# Autodesk Inventor assembly: 046-DXP(F,D-166-3)
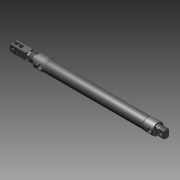
[picture p0: Inventor's stored thumbnail of the model, 180x180]
Saved by Autodesk Inventor 2015 (Build 190159000, 159)
## iProperties
Category: PARTsolutions
Company: BIMBA
Created: 2015-01-31
Part Number: 046-DXP(F,D-166-3)
Catalog Web Link: www.cadenas.de
Description: Original Line Standard Air Cylinders-
Vendor: BIMBA
Document SubType Name: Assembly
Designer: PARTuser1
Manufacturer: BIMBA
PSOL_IDENT_0: {$CADENAS_DATA\23d-libs\bimba\bimba\bimba_imperial\bimba_full_line\original_line_cylinders\standard_
PSOL_IDENT_1: air_cylinders\standard_air_cylinder_asmtab.prj},325 {VTYP=3D},{STYP=ASSTAB},{NB=046-DXP(F,D-166-3)},
PSOL_IDENT_2: {LINA=046-DXP},{NN=Original Line Standard Air Cylinders},{DATE=08.09.2014 04:47:41},{GEOMDATE=08.09.
PSOL_IDENT_3: 2014 04:47:39},{VERSION=},{LINEID=50},{LINESUBID=-1},{WBVAR=STROKE,ACTING,MNT,DER,NR,BM,CO,OO,VO,M,E
PSOL_IDENT_4: E,EEL,K,Q,Y,G,T,B,H,SER,SR,NT,W,HL,STPT1,STPT2,STPT3,STPT4,MB,PB,PRC,TB,MN}  {NB=046-DXP(F,D-166-3)}
PSOL_IDENT_5: ,{LINA=046-DXP},{KT=DUMMY},{PN=046-DXP},{PNC=046-DXP(F,D-166-3)},{PNA=(D-166-3)},{DASH=-},{BORE1=0.7
PSOL_IDENT_6: 5000000},{BORE=3/4\" (04)},{BOREPN=04},{STROKE=6.000},{STROKEALG=[0.011:50/0.001]},{STROKE1=6.000},{
PSOL_IDENT_7: ACTING=D},{ACTINGALG= '' , 'Single Acting (SA)' , 'R' , 'Reverse Single Acting (SA)' , 'D' , 'Double
PSOL_IDENT_8: Acting (SA)' },{ACTINGPN=D},{MNT=XP},{MNTALG= '' , 'Front Nose Mounting (SA)' , 'P' , 'Rear Pivot M
PSOL_IDENT_9: ounting (SA)' , 'XP' , 'Double End or Pivot Mounting (SA)' , 'X' , 'Double End Mounting (SA)' , 'BF'
PSOL_IDENT_10: , 'Front Block Mounting (SA)' , 'BR' , 'Rear Block Mounting for Vertical Positioning (SA)' , 'BFT'
PSOL_IDENT_11: , 'Front Block Trunnion Mounting (SA)' , 'BRT' , 'Rear Block Trunnion Mounting (SA)' },{TYPE=},{MNTP
PSOL_IDENT_12: N=XP},{DER=},{DERALG= '' , 'N/A' },{NR=},{NRALG= '' , 'N/A' },{NRPN=},{BM=},{BMALG= '' , 'N/A' },{BM
PSOL_IDENT_13: PN=},{CO=},{COALG= '' , 'N/A' },{OO=},{OOALG= '', 'N/A' },{OOPN=},{VO=Z},{VOALG= 'Z' , 'N/A' },{VOPN=
PSOL_IDENT_14: },{OOVOPN=},{M=},{MALG= '', 'Without Magnet', 'M', 'With Magnet' },{EE=},{EEL=0.000},{EEMAX=44.0000}
PSOL_IDENT_15: ,{EEALG= '', 'Without Extra Extension', 'EE', 'With Extra Extension' },{EELALG=0},{EEPN=},{EEPN1=0.0
PSOL_IDENT_16: 00},{K=},{KALG= '', 'Standard' , 'K' , 'Ports Rotated 90deg K' },{KPN=},{Q=},{QALG= '' , 'N/A' },{QP
PSOL_IDENT_17: N=},{Y=},{YALG= '' , 'Without Pivot Bushing' , 'Y' , 'With Pivot Bushing' },{YPN=},{YCON=},{F=},{FAL
PSOL_IDENT_18: G= '', 'Non-Coated (Standard)', 'F', 'Molycoated' },{FPN=},{G=},{GPN=},{GPN99=},{T=},{TALG= '' , 'St
PSOL_IDENT_19: andard -20° to 200°F (-29° to 95°C)' , 'N' , 'Low Temperature' , 'V' , 'High Temperature' },{NPN=},{
PSOL_IDENT_20: VPN=},{B=},{BALG= '', 'W/out Bumpers' , 'B' , 'W/ Bumpers' },{BPN=},{H=},{HALG= '', 'N/A' },{HPN=},{
PSOL_IDENT_21: SER=},{SERALG= '' , 'Without Spring Extend/Return' , 'JS' , 'With Spring Return' , 'JR' , 'With Spri
PSOL_IDENT_22: ng Extend' },{SR=},{SRALG= '' , 'Standard Stainless Steel' },{SRPN=},{SRCON=0},{NT=},{NTPN=},{W=},{W
PSOL_IDENT_23: ALG= '' , 'Without Wiper' , 'W' , 'With Wiper' },{WPN=},{E=},{EALG= '' , 'Standard Seals/Lube' , 'E'
PSOL_IDENT_24: , 'Non-Lube Seals/Lube' },{EPN=},{HL=},{HLALG= '' , 'Without Low Pressure Hydraulic' , 'HL' , 'With
PSOL_IDENT_25: Low Pressure Hydraulic' },{ST=},{STALG= '' , 'N/A' },{STPT1=},{STPT1ALG= '' , 'N/A' },{STPT2=},{STP
PSOL_IDENT_26: T2ALG= '' , 'N/A' },{STPT3=},{STPT3ALG= '' , 'N/A' },{STPT4=},{STPT4ALG= '' , 'N/A' },{STPN=},{MB=},
PSOL_IDENT_27: {MBALG= '' , 'Without Mounting Bracket' , 'F,D-129' , 'D-129 (front)'  , 'R,D-129' , 'D-129 (rear)'
PSOL_IDENT_28: , '2x,D-129' , 'D-129 (front & rear)'},{MBPN=},{MBPNALL=D-129},{MBPNALLREAR=D-129},{PB=},{PBALG= ''
PSOL_IDENT_29: , 'Without Pivot Bracket' , 'D-13498-A' , 'D-13498-A' },{PBPN=},{PBPNALL=D-13498-A},{PRC=F,D-166-3},
PSOL_IDENT_30: {PRCALG= '' , 'W/out Pivot Rod Clevis' , 'F,D-166-3' , 'D-166-3 (front)' },{PRCPN=(F,D-166-3)},{PRCP
PSOL_IDENT_31: NALL=D-166-3},{TB=},{TBALG= '' , 'N/A' },{TBPN=},{TBPNALL=},{MN=},{MNALG= '' , 'N/A' },{MNPN=},{MNCO
PSOL_IDENT_32: NF=},{MNCONR=},{TLEN=7.2555},{FRAC=44.7500},{RGCON=},{RGDACCON=R},{RHCON=P},{RHCON1=P},{RHCONON=1},{
PSOL_IDENT_33: RHACCON=},{FNUTCON=1},{RNUTCON=1},{FNUTPN=D-9},{RNUTPN=D-9},{FNUTTRANS=0.0000},{RNUTTRANS=0.0000},{V
PSOL_IDENT_34: HOLECON=0},{A1=1.5940},{A1N=0.8750},{A1P=1.5940},{A1B=1.5940},{A4=0.2525},{A4N=0.3130},{A4P=0.2525},
PSOL_IDENT_35: {A5=0.0300},{A1H=1.594},{A1NH=0.5310},{A1PH=1.5940},{A1BH=1.0940},{A1SH=1.2190},{A2H=0.2190},{A2NH=0
PSOL_IDENT_36: .2190},{LENGTH=3.7500},{LENGTH1=3.7500},{LENGTH2=3.8100},{MUL=6.0000},{MUL11=6.0000},{MUL22=16.14},{
PSOL_IDENT_37: MUL33=10.1400},{MUL2=6.0000},{MUL211=6.0000},{MUL222=2.6900},{MUL233=1.6900},{SSS=12.0000},{RGLEN=1.
PSOL_IDENT_38: 3715},{RHLEN=1.1230},{SSS1=7.0000},{A13=1.3120},{DIF=0.0000},{G5=0.6250},{ON=0},{SSADD=0.0000},{BADD=
PSOL_IDENT_39: 0.0000},{MADD=0.0000},{NVADD=0.0000},{TRACKL=6.9655},{TRACKCON=D-74168},{TRIMCON=0},{TRIMCON1=0},{PI
PSOL_IDENT_40: NCON=D-51},{FSPACE=0.7783},{SPACE=0.1071},{TEXT=0.1875},{S1=1.0000},{D1=0.8325},{D1N=0.8050},{D1B=0.
PSOL_IDENT_41: 8625},{D1P=0.8325},{FA=0.940},{RA=0.9400},{PPATH=standard_air_cylinder_asmtpl.prj},{MATALGHTML=<b>St
PSOL_IDENT_42: andard Original Line:</b><dl><dt>Rod:</dt><dd>- Stainless Steel</dd><dd>&nbsp;&nbsp;(5/16 9/16 Bores
PSOL_IDENT_43: )</dd><dd>- High Strength Carbon Steel</dd><dd>&nbsp;&nbsp;(3/4 3 Bore)</dd><dd>- Stainless Steel</d
PSOL_IDENT_44: d><dd>&nbsp;&nbsp;(X style DXP/DX/DXDE)</dd><dt>Bearings:</dt><dd>- Sintered Bronze</dd><dt>Body:</d
PSOL_IDENT_45: t><dd>- 304 Stainless Steel</dd><dt>End Caps:</dt><dd>- Aluminum</dd><dt>Seals:</dt><dd>- Buna N</dd
PSOL_IDENT_46: ></dl>},{ASSCFGPRA=04DXP},{MBPNA=},{MNPNA=},{PRCPNA=(D-166-3)},{ASSOPTACC=STPT4},{A=9.75},{HADD=0.00
PSOL_IDENT_47: 00},{WFL=0.25},{QADD=0.000},{QADD1=0.440},{TEST=6.0000},{MNTB=},{STDNUTF=1},{STDNUTR=1}
SUPPLIER: BIMBA
ARTICLENO: 046-DXP(F,D-166-3)
BOMINFO: 046-DXP
CREATOR: CADENAS GmbH
Title: 046-DXP
Author: Cadenas PARTsolutions
## Documents named in this file (11)
- C:\Users\Brian\Documents\GitHub\FIRST-Team-1719-CAD-Team\2015 Robot CAD\Brian's Practice\Piston\Piston.iam
- C:\Users\Brian\Documents\GitHub\FIRST-Team-1719-CAD-Team\2015 Robot CAD\Brian's Practice\Piston\046_DXP_F_D_166_3_0000_0_dummy.ipt
- C:\Users\Brian\Documents\GitHub\FIRST-Team-1719-CAD-Team\2015 Robot CAD\Brian's Practice\Piston\04R000_0_rod_guide.ipt
- C:\Users\Brian\Documents\GitHub\FIRST-Team-1719-CAD-Team\2015 Robot CAD\Brian's Practice\Piston\04R_7_25550.ipt
- C:\Users\Brian\Documents\GitHub\FIRST-Team-1719-CAD-Team\2015 Robot CAD\Brian's Practice\Piston\04P0000_rear_head.ipt
- C:\Users\Brian\Documents\GitHub\FIRST-Team-1719-CAD-Team\2015 Robot CAD\Brian's Practice\Piston\046_DXP0_rod.ipt
- C:\Users\Brian\Documents\GitHub\FIRST-Team-1719-CAD-Team\2015 Robot CAD\Brian's Practice\Piston\D_166_3_dummy.ipt
- C:\Users\Brian\Documents\GitHub\FIRST-Team-1719-CAD-Team\2015 Robot CAD\Brian's Practice\Piston\D_14055.ipt
- C:\Users\Brian\Documents\GitHub\FIRST-Team-1719-CAD-Team\2015 Robot CAD\Brian's Practice\Piston\D_8381.ipt
- C:\Users\Brian\Documents\GitHub\FIRST-Team-1719-CAD-Team\2015 Robot CAD\Brian's Practice\Piston\D_5866.ipt
- C:\Users\Brian\Documents\GitHub\FIRST-Team-1719-CAD-Team\2015 Robot CAD\Brian's Practice\Piston\D_344.ipt
## Components (11 placed, 10 different names)
1. 046_DXP_F_D_166_3_0000_0_dummy:1
2. 04R000_0_rod_guide:1 — Mate:9
3. 04R_7_25550:1
4. 04P0000_rear_head:1 — Angle:3
5. 046_DXP0_rod:1 — Mate:7, Flush:3, Mate:9
6. D_166_3_dummy:1
7. D_14055:1 — Mate:1, Mate:4, Flush:2, Mate:5, Angle:1, Angle:2, Mate:6, Mate:7, Mate:8, Flush:3, Angle:3
8. D_8381:1 — Mate:2, Mate:3, Flush:2, Mate:5
9. D_5866:1 — Mate:1, Mate:2, Flush:1
10. D_5866:2 — Flush:1, Mate:3, Mate:4, Angle:1
11. D_344:1 — Angle:2, Mate:6, Mate:8
## Relationships (15: Mate 9, Flush 3, Angle 3)
- Mate:1: D_14055:1 ↔ D_5866:1
- Mate:2: D_8381:1 ↔ D_5866:1
- Flush:1: D_5866:1 ↔ D_5866:2
- Mate:3: D_8381:1 ↔ D_5866:2
- Mate:4: D_14055:1 ↔ D_5866:2
- Flush:2 (-2.413 mm): D_14055:1 ↔ D_8381:1
- Mate:5: D_14055:1 ↔ D_8381:1
- Angle:1 (60 deg): D_14055:1 ↔ D_5866:2
- Angle:2 (30 deg): D_14055:1 ↔ D_344:1
- Mate:6: D_14055:1 ↔ D_344:1
- Mate:7: 046_DXP0_rod:1 ↔ D_14055:1
- Mate:8: D_14055:1 ↔ D_344:1
- Flush:3 (4.064 mm): 046_DXP0_rod:1 ↔ D_14055:1
- Mate:9: 04R000_0_rod_guide:1 ↔ 046_DXP0_rod:1
- Angle:3 (0 deg): 04P0000_rear_head:1 ↔ D_14055:1
